# Autodesk Inventor assembly: WCD V2
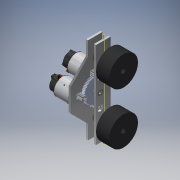
[picture p0: Inventor's stored thumbnail of the model, 180x180]
Saved by Autodesk Inventor 2019.4 (Build 234330000, 330)
## iProperties
Created: 2019-12-07
Part Number: WCD V2
Document SubType Name: Assembly
Designer: admin
Mass: 3479.8 g
Surface Area: 4188.3 cm^2
Volume: 1585.96 cm^3
Density: 2.19414 g/cm^3
Author: admin
## Documents named in this file (9)
- C:\Users\Mark\Desktop\7738 Helion Engineering\7738-CAD-prep\WCD\WCD V2.iam
- C:\Users\Mark\Desktop\7738 Helion Engineering\7738-CAD-prep\Swerve Module\Falcon_500_Powered_by_Talon_FX_217-6515.iam
- C:\Users\Mark\Desktop\7738 Helion Engineering\7738-CAD-prep\WCD\10T_Steel_Spur_Gear_20_DP_12T_Center_Distance_Falcon_Motor_217-6917.ipt
- C:\Users\Mark\Desktop\7738 Helion Engineering\7738-CAD-prep\WCD\Wheel.ipt
- C:\Users\Mark\Desktop\7738 Helion Engineering\7738-CAD-prep\WCD\Inner Plate.ipt
- C:\Users\Mark\Desktop\7738 Helion Engineering\7738-CAD-prep\WCD\Outer Plate.ipt
- C:\Users\Mark\Desktop\7738 Helion Engineering\7738-CAD-prep\WCD\64t_Aluminum_Spur_Gear_20_DP_1_2_Hex_Bore_217-3575.ipt
- C:\Users\Mark\Desktop\7738 Helion Engineering\7738-CAD-prep\WCD\F6902zz.ipt
- C:\Users\Mark\Desktop\7738 Helion Engineering\7738-CAD-prep\WCD\F63800.ipt
## Components (17 placed, 8 different names)
1. Wheel:1 — Flush:7, Mate:43
2. Wheel:2 — Flush:7, Mate:41, Mate:42
3. OutPlate — Flush:9, Mate:39, Mate:40, Mate:41, Mate:42, Mate:43, Mate:46, Mate:47, Mate:48, Mate:49, Mate:52, Mate:53
4. InPlate — Mate:23, Mate:24, Mate:27, Mate:28, Mate:29, Mate:30, Mate:31, Mate:33, Mate:35, Mate:37, Mate:38, Flush:9, Mate:39, Mate:40, Mate:44, Mate:45, Mate:50, Mate:51, Mate:54, Mate:55
5. F63800:1 — Mate:52, Mate:53
6. F63800:2 — Mate:54, Mate:55
7. Falcon_500_Powered_by_Talon_FX_217-6515:1 [sub-assembly] — Mate:23, Mate:27, Mate:34
8. Falcon_500_Powered_by_Talon_FX_217-6515:2 [sub-assembly] — Mate:24, Mate:28, Mate:36
9. Falcon_500_Powered_by_Talon_FX_217-6515:3 [sub-assembly] — Mate:29, Mate:30, Mate:32
10. 64t_Aluminum_Spur_Gear_20_DP_1_2_Hex_Bore_217-3575:1 — Mate:31, Mate:38
11. 10T_Steel_Spur_Gear_20_DP_12T_Center_Distance_Falcon_Motor_217-6917:1 — Mate:32, Mate:33
12. 10T_Steel_Spur_Gear_20_DP_12T_Center_Distance_Falcon_Motor_217-6917:2 — Mate:34, Mate:35
13. 10T_Steel_Spur_Gear_20_DP_12T_Center_Distance_Falcon_Motor_217-6917:3 — Mate:36, Mate:37
14. F6902zz:2 — Mate:50, Mate:51
15. F6902zz:3 — Mate:46, Mate:47
16. F6902zz:4 — Mate:48, Mate:49
17. F6902zz:1 — Mate:44, Mate:45
## Relationships (34: Mate 31, Flush 3)
- Flush:7: Wheel:1 ↔ Wheel:2
- Flush:8 (20 mm)
- Mate:23: InPlate ↔ Falcon_500_Powered_by_Talon_FX_217-6515:1
- Mate:24: InPlate ↔ Falcon_500_Powered_by_Talon_FX_217-6515:2
- Mate:27: InPlate ↔ Falcon_500_Powered_by_Talon_FX_217-6515:1
- Mate:28: InPlate ↔ Falcon_500_Powered_by_Talon_FX_217-6515:2
- Mate:29: InPlate ↔ Falcon_500_Powered_by_Talon_FX_217-6515:3
- Mate:30: InPlate ↔ Falcon_500_Powered_by_Talon_FX_217-6515:3
- Mate:31: InPlate ↔ 64t_Aluminum_Spur_Gear_20_DP_1_2_Hex_Bore_217-3575:1
- Mate:32: Falcon_500_Powered_by_Talon_FX_217-6515:3 ↔ 10T_Steel_Spur_Gear_20_DP_12T_Center_Distance_Falcon_Motor_217-6917:1
- Mate:33: InPlate ↔ 10T_Steel_Spur_Gear_20_DP_12T_Center_Distance_Falcon_Motor_217-6917:1
- Mate:34: Falcon_500_Powered_by_Talon_FX_217-6515:1 ↔ 10T_Steel_Spur_Gear_20_DP_12T_Center_Distance_Falcon_Motor_217-6917:2
- Mate:35: InPlate ↔ 10T_Steel_Spur_Gear_20_DP_12T_Center_Distance_Falcon_Motor_217-6917:2
- Mate:36: Falcon_500_Powered_by_Talon_FX_217-6515:2 ↔ 10T_Steel_Spur_Gear_20_DP_12T_Center_Distance_Falcon_Motor_217-6917:3
- Mate:37: InPlate ↔ 10T_Steel_Spur_Gear_20_DP_12T_Center_Distance_Falcon_Motor_217-6917:3
- Mate:38 (3 mm): InPlate ↔ 64t_Aluminum_Spur_Gear_20_DP_1_2_Hex_Bore_217-3575:1
- Flush:9: OutPlate ↔ InPlate
- Mate:39: OutPlate ↔ InPlate
- Mate:40 (21 mm): OutPlate ↔ InPlate
- Mate:41: Wheel:2 ↔ OutPlate
- Mate:42 (20 mm): Wheel:2 ↔ OutPlate
- Mate:43: Wheel:1 ↔ OutPlate
- Mate:44: InPlate ↔ F6902zz:1
- Mate:45: InPlate ↔ F6902zz:1
- Mate:46: OutPlate ↔ F6902zz:3
- Mate:47: OutPlate ↔ F6902zz:3
- Mate:48: OutPlate ↔ F6902zz:4
- Mate:49: OutPlate ↔ F6902zz:4
- Mate:50: InPlate ↔ F6902zz:2
- Mate:51: InPlate ↔ F6902zz:2
- Mate:52: OutPlate ↔ F63800:1
- Mate:53: OutPlate ↔ F63800:1
- Mate:54: InPlate ↔ F63800:2
- Mate:55: InPlate ↔ F63800:2
